# Autodesk Inventor assembly: 知能ロボコン合体１
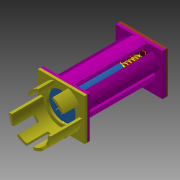
[picture p0: Inventor's stored thumbnail of the model, 180x180]
Saved by Autodesk Inventor 2013 (Build 170138000, 138)
## iProperties
Created: 2014-05-17
Part Number: 知能ロボコン合体１
Document SubType Name: Assembly
Designer: horumo136
Author: horumo136
## Documents named in this file (8)
- C:\Users\horumo136\Documents\知能ロボコン合体１.iam
- C:\Users\horumo136\Documents\知能ロボコン発射口.ipt
- C:\Users\horumo136\Documents\知能ロボコン外筒.ipt
- C:\Users\horumo136\Documents\知能ロボコンシリンダ.ipt
- C:\Users\horumo136\Documents\知能ロボコンラックギア.ipt
- C:\Users\horumo136\Documents\知能ロボコンばね112038.ipt
- C:\Users\horumo136\Documents\知能ロボコンばね受け.ipt
- C:\Users\horumo136\Documents\知能ロボコンばね受け受け.ipt
## Components (7 placed, 7 different names)
1. 知能ロボコン発射口:1
2. 知能ロボコン外筒:1 — メイト:15, 挿入:1, メイト:26
3. 知能ロボコンシリンダ:1 — メイト:10, メイト:12, メイト:14, メイト:15
4. 知能ロボコンラックギア:1 — メイト:10, メイト:12, メイト:14
5. 知能ロボコンばね112038:1 — メイト:19, メイト:20, メイト:21
6. 知能ロボコンばね受け:1 — メイト:19, メイト:20, メイト:21, 挿入:1
7. 知能ロボコンばね受け受け:1 — メイト:26
## Relationships (9: Mate 8, Insert 1)
- メイト:10 [Mate]: 知能ロボコンシリンダ:1 ↔ 知能ロボコンラックギア:1
- メイト:12 [Mate]: 知能ロボコンシリンダ:1 ↔ 知能ロボコンラックギア:1
- メイト:14 [Mate]: 知能ロボコンシリンダ:1 ↔ 知能ロボコンラックギア:1
- メイト:15 [Mate]: 知能ロボコン外筒:1 ↔ 知能ロボコンシリンダ:1
- メイト:19 [Mate]: 知能ロボコンばね112038:1 ↔ 知能ロボコンばね受け:1
- メイト:20 [Mate]: 知能ロボコンばね112038:1 ↔ 知能ロボコンばね受け:1
- メイト:21 [Mate]: 知能ロボコンばね112038:1 ↔ 知能ロボコンばね受け:1
- 挿入:1 [Insert]: 知能ロボコン外筒:1 ↔ 知能ロボコンばね受け:1
- メイト:26 [Mate]: 知能ロボコン外筒:1 ↔ 知能ロボコンばね受け受け:1
